# Autodesk Inventor assembly: cabinet_assembly
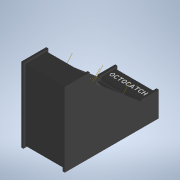
[picture p0: Inventor's stored thumbnail of the model, 180x180]
Saved by Autodesk Inventor 2020 (Build 240168000, 168)
## iProperties
Created: 2021-03-06
Part Number: cabinet_assembly
Document SubType Name: Assembly
Designer: Harry
Author: Harry
## Documents named in this file (5)
- C:\Users\Harry\Documents\hacktheburgh\octocatch\cad\cabinet_assembly.iam
- C:\Users\Harry\Documents\hacktheburgh\octocatch\cad\cabinet.ipt
- C:\Users\Harry\Documents\hacktheburgh\octocatch\cad\main_assembly.iam
- C:\Users\Harry\Documents\hacktheburgh\octocatch\cad\20 pixel strip.iam
- C:\Users\Harry\Documents\hacktheburgh\octocatch\cad\20 pixel strip_MIR.iam
## Components (4 placed, 4 different names)
1. cabinet:1 — Mate:1, Mate:2, Mate:3, Mate:4, Mate:5
2. main_assembly:1 [sub-assembly] — Mate:1, Mate:2, Mate:3
3. 20 pixel strip:1 [sub-assembly] — Mate:4, Mate:5
4. 20 pixel strip_MIR:1 [sub-assembly]
## Relationships (5: Mate 5)
- Mate:1: cabinet:1 ↔ main_assembly:1
- Mate:2: cabinet:1 ↔ main_assembly:1
- Mate:3: cabinet:1 ↔ main_assembly:1
- Mate:4: cabinet:1 ↔ 20 pixel strip:1
- Mate:5 (20 mm): cabinet:1 ↔ 20 pixel strip:1
